# Autodesk Inventor assembly: GSHCCGH6-52.0
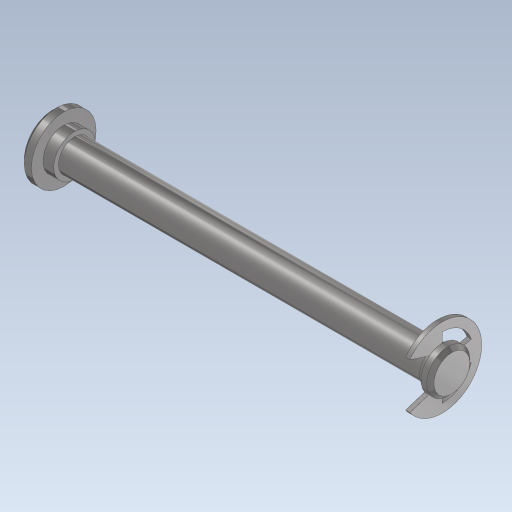
[picture p0: Inventor's stored thumbnail of the model, 512x512]
Saved by Autodesk Inventor 2024 (Build 280153000, 153)
## iProperties
Created: 2023-10-14
Part Number: GSHCCGH6-52.0
Catalog Web Link: www.cadenas.de
Description: HCCG, HCCGH, PHCCG, PHCCGH, GHCCG, SHCCG, SHCCGH, GSHCCGH-Hinge Pins - Retaining Ring Type with Shoulder - L Dimension Specified Type (0.1mm Increment)
Vendor: MISUMI
Document SubType Name: Assembly
Designer: psAdmin
Manufacturer: MISUMI
Mass: 13.0677 g
Surface Area: 13.1081 cm^2
Volume: 1.63347 cm^3
Density: 8 g/cm^3
Category: PARTsolutions
Company: MISUMI
PSOL_IDENT_0: {$CADENAS_DATA/23d-libs/misumi/metric/13_cantilever_shafts/hccg_asmtab.prj},285 {VTYP=3D},{STYP=ASST
PSOL_IDENT_1: AB},{NB=GSHCCGH6-52.0},{LINA=GSHCCGH6-52.0},{NN=HCCG, HCCGH, PHCCG, PHCCGH, GHCCG, SHCCG, SHCCGH, GS
PSOL_IDENT_2: HCCGH},{DATE=21.04.2022 08:37:14},{GEOMDATE=17.06.2021 11:01:05},{VERSION=},{LINEID=40},{WBVAR=MAT,H
PSOL_IDENT_3: ARD,ST,L,ALT1,NC,ALT2,TC,ALT3,ALT4,TBH},{WBNUMERIC=L,NC,TC,TBH}  {NB=GSHCCGH6-52.0},{LINA=GSHCCGH6-5
PSOL_IDENT_4: 2.0},{KT=DUMMY},{PN=GSHCCGH6-52.0},{TYPE=GSHCCGH},{MAT=3},{HARD=5},{HARD1= '4','45~50HRC','5','45~50
PSOL_IDENT_5: HRC Plating Hardness 750HV~' },{ST=4},{ST1='4','Hard Chrome Plating'},{AC=Retaining Ring 1 pc.},{MAT
PSOL_IDENT_6: AC=SUS304},{D=6},{DTOL=-0.004/-0.012},{L=52.0},{LS1=[5.0-120.0/0.1]},{L2=52},{L3=0},{LPN=52.0},{M=0.
PSOL_IDENT_7: 70},{MTOL=+0.1/0},{ALT1=},{NC=0.0},{N=2},{N1=2},{NC1=[1.9-4.0/0.1]},{NC2=0},{NC3=0},{NC4=0},{NCPN=0.
PSOL_IDENT_8: 0},{ALT1PN=},{UU=5.8},{NN=1.5},{DD=5.0},{DDTOL=+0.075/0},{ALT2=},{TC=0.0},{T=1.5},{TT1=1.5},{TC1=0},
PSOL_IDENT_9: {TMIN=2},{TC2=0},{TC3=0},{TCT=0.0},{ALT2PN=},{H=9.0},{RRS=E Type},{RRN=No.5},{PPATH=hccg_templ.prj},
PSOL_IDENT_10: {ALT3=},{HC=3.50},{ALT4=},{ALT4ALG= '', 'w/o TBH (Shoulder Diameter)', '-TBH', 'with TBH (Shoulder D
PSOL_IDENT_11: iameter)' },{TBH=0.0},{TBHALG=0},{TBHMIN=7.0},{TBHMAX=8.5},{H3D=9.0},{ALT4PN=}
NB: GSHCCGH6-52.0
NN: 1.5
NT: Hinge Pins - Retaining Ring Type with Shoulder - L Dimension Specified Type (0.1mm Increment)
NBSYN: $PN.
LINA: GSHCCGH6-52.0
CATALOG: Misumi
PN: GSHCCGH6-52.0
MAT: SUS440C or 13Cr Stainless Steel
HARD: 45~50HRC Plating Hardness 750HV~
ST: Hard Chrome Plating
MATAC: SUS304
D: 6
L: 52
M: 0.7
MTOL: +0.1/0
ALT1: w/o NC (Retaining Ring Groove Position)
NC: 0
N: 2
UU: 5.8
DD: 5
DDTOL: +0.075/0
ALT2: w/o TC (Shoulder Thickness)
TC: 0
T: 1.5
H: 9
RRS: E Type
RRN: No.5
ALT3: w/o HC (Shoulder Diameter Cut)
ALT4: w/o TBH (Shoulder Diameter)
TBH: 0
SUPPLIER: MISUMI
ARTICLENO: GSHCCGH6-52.0
BOMINFO: GSHCCGH6-52.0
CREATOR: CADENAS GmbH
Title: GSHCCGH6-52.0
Author: Cadenas PARTsolutions
Comments: Hinge Pins - Retaining Ring Type with Shoulder - L Dimension Specified Type (0.1mm Increment)
## Documents named in this file (3)
- C:\Users\michi\OneDrive - Kyoto University\lab\6_SHINOBI\FUHGA4\Design_Mechanism\05_birdeye\birdeye_elbowUnit\GSHCCGH6-52_Autodesk_Inventor_2024_20231014\AIS2024\GSHCCGH6-52_0.iam
- C:\Users\michi\OneDrive - Kyoto University\lab\6_SHINOBI\FUHGA4\Design_Mechanism\05_birdeye\birdeye_elbowUnit\GSHCCGH6-52_Autodesk_Inventor_2024_20231014\AIS2024\GSHCCGH6-52_0_D.ipt
- C:\Users\michi\OneDrive - Kyoto University\lab\6_SHINOBI\FUHGA4\Design_Mechanism\05_birdeye\birdeye_elbowUnit\GSHCCGH6-52_Autodesk_Inventor_2024_20231014\AIS2024\RRING_E_EXT-S-5.ipt
## Components (2 placed, 2 different names)
1. GSHCCGH6-52_0_D:1 — pin_to_rring_XY@1 <-> ring_to_screw_XY@2, pin_to_rring_Z@1 <-> ring_to_screw_Z@2, pin_to_rring_YZ@1 <-> ring_to_screw_YZ@2
2. RRING_E_EXT-S-5:1 — pin_to_rring_XY@1 <-> ring_to_screw_XY@2, pin_to_rring_Z@1 <-> ring_to_screw_Z@2, pin_to_rring_YZ@1 <-> ring_to_screw_YZ@2
## Relationships (3: Mate 2, Angle 1)
- pin_to_rring_XY@1 <-> ring_to_screw_XY@2 [Mate]: GSHCCGH6-52_0_D:1 ↔ RRING_E_EXT-S-5:1
- pin_to_rring_Z@1 <-> ring_to_screw_Z@2 [Mate]: GSHCCGH6-52_0_D:1 ↔ RRING_E_EXT-S-5:1
- pin_to_rring_YZ@1 <-> ring_to_screw_YZ@2 [Angle] (0 deg): GSHCCGH6-52_0_D:1 ↔ RRING_E_EXT-S-5:1
